# Autodesk Inventor assembly: buoy_mainboard
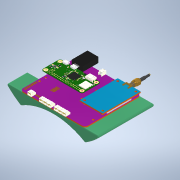
[picture p0: Inventor's stored thumbnail of the model, 180x180]
Saved by Autodesk Inventor 2020.2 (Build 242310000, 310)
## iProperties
Created: 2020-04-10
Part Number: buoy_mainboard
Document SubType Name: Assembly
Designer: agmlego
Mass: 108.257 g
Surface Area: 767.177 cm^2
Volume: 137.886 cm^3
Density: 0.785117 g/cm^3
Author: agmlego
## Documents named in this file (10)
- D:\projects\CreekFleet_AutoBuoy\Mechanical CAD\controls\buoy_mainboard.iam
- D:\projects\CreekFleet_AutoBuoy\Mechanical CAD\controls\buoy_pcb.ipt
- D:\projects\CreekFleet_AutoBuoy\Mechanical CAD\controls\pi-zero\RapberryPiZero.iam
- D:\projects\CreekFleet_AutoBuoy\Mechanical CAD\controls\XT09-SI.ipt
- D:\projects\CreekFleet_AutoBuoy\Mechanical CAD\controls\JST-PH-2\S2B-PH-K-S(LF)(SN)--3DModel-STEP-1.ipt
- D:\projects\CreekFleet_AutoBuoy\Mechanical CAD\controls\ND-105C.ipt
- D:\projects\CreekFleet_AutoBuoy\Mechanical CAD\controls\pololu\dual-g2-hpmd-18v18-24v14-raspberry-pi.ipt
- D:\projects\CreekFleet_AutoBuoy\Mechanical CAD\controls\mainboard_mount.ipt
- D:\projects\CreekFleet_AutoBuoy\Mechanical CAD\94459A140_BRASS HEAT-SET INSERT FOR PLASTIC.ipt
- D:\projects\CreekFleet_AutoBuoy\Mechanical CAD\controls\rp-sma_end.ipt
## Components (21 placed, 16 different names)
1. buoy_pcb:1 — Mate:1, Flush:1, Flush:2, Mate:2, Mate:3, Mate:4, Mate:5, Mate:6, Mate:7, Mate:8, Mate:9, Mate:10, Mate:11, Mate:12, Mate:13, Mate:14, Mate:15, Tangent:1, Tangent:2, Tangent:3, Tangent:4, Tangent:5, Tangent:6, Tangent:7, Tangent:8, Tangent:9, Tangent:10, Tangent:11, Tangent:12, Mate:19, Mate:20, Mate:21, Insert:1, Angle:1
2. RapberryPiZero:1 [sub-assembly] — Mate:2, Mate:3, Mate:4, Mate:16, Mate:17, Mate:18
3. XT09-SI:1 — Mate:5, Mate:6, Mate:7, Insert:8
4. CAN — Mate:15, Tangent:1, Tangent:2, Tangent:3
5. CURR — Mate:8, Flush:8, Tangent:4, Tangent:12
6. FLT — Mate:9, Flush:7, Flush:8, Tangent:11
7. SLP — Mate:10, Flush:6, Flush:7, Tangent:10
8. DIR — Mate:11, Flush:5, Flush:6, Tangent:9
9. PORT LED — Mate:12, Flush:4, Flush:5, Tangent:8
10. STAR LED — Mate:13, Flush:3, Flush:4, Tangent:7
11. ALLROUND LED — Mate:14, Flush:3, Tangent:5, Tangent:6
12. ND-105C:1 — Mate:16, Mate:17, Mate:18
13. dual-g2-hpmd-18v18-24v14-raspberry-pi:1 — Mate:19, Mate:20, Mate:21
14. mainboard_mount:1 — Insert:1, Angle:1, Insert:2, Insert:3, Insert:4, Insert:5, Insert:6, Insert:7
15. 94459A140_BRASS HEAT-SET INSERT FOR PLASTIC:1 — Insert:2
16. 94459A140_BRASS HEAT-SET INSERT FOR PLASTIC:2 — Insert:3
17. 94459A140_BRASS HEAT-SET INSERT FOR PLASTIC:3 — Insert:4
18. 94459A140_BRASS HEAT-SET INSERT FOR PLASTIC:4 — Insert:5
19. 94459A140_BRASS HEAT-SET INSERT FOR PLASTIC:5 — Insert:7
20. 94459A140_BRASS HEAT-SET INSERT FOR PLASTIC:6 — Insert:6
21. rp-sma_end:1 — Insert:8
## Relationships (50: Mate 21, Tangent 12, Flush 8, Insert 8, Angle 1)
- Mate:1: buoy_pcb:1
- Flush:1: buoy_pcb:1
- Flush:2: buoy_pcb:1
- Mate:2: buoy_pcb:1 ↔ RapberryPiZero:1
- Mate:3: buoy_pcb:1 ↔ RapberryPiZero:1
- Mate:4 (10 mm): buoy_pcb:1 ↔ RapberryPiZero:1
- Mate:5: buoy_pcb:1 ↔ XT09-SI:1
- Mate:6: buoy_pcb:1 ↔ XT09-SI:1
- Mate:7: buoy_pcb:1 ↔ XT09-SI:1
- Mate:8: buoy_pcb:1 ↔ CURR
- Mate:9: buoy_pcb:1 ↔ FLT
- Mate:10: buoy_pcb:1 ↔ SLP
- Mate:11: buoy_pcb:1 ↔ DIR
- Mate:12: buoy_pcb:1 ↔ PORT LED
- Mate:13: buoy_pcb:1 ↔ STAR LED
- Mate:14: buoy_pcb:1 ↔ ALLROUND LED
- Mate:15: buoy_pcb:1 ↔ CAN
- Tangent:1: buoy_pcb:1 ↔ CAN
- Tangent:2: buoy_pcb:1 ↔ CAN
- Tangent:3 (0.6 mm): buoy_pcb:1 ↔ CAN
- Flush:3: STAR LED ↔ ALLROUND LED
- Flush:4: PORT LED ↔ STAR LED
- Flush:5: DIR ↔ PORT LED
- Flush:6: SLP ↔ DIR
- Flush:7: FLT ↔ SLP
- Flush:8: CURR ↔ FLT
- Tangent:4: buoy_pcb:1 ↔ CURR
- Tangent:5: buoy_pcb:1 ↔ ALLROUND LED
- Tangent:6 (0.6 mm): buoy_pcb:1 ↔ ALLROUND LED
- Tangent:7 (0.6 mm): buoy_pcb:1 ↔ STAR LED
- Tangent:8 (0.6 mm): buoy_pcb:1 ↔ PORT LED
- Tangent:9 (0.6 mm): buoy_pcb:1 ↔ DIR
- Tangent:10 (0.6 mm): buoy_pcb:1 ↔ SLP
- Tangent:11 (0.6 mm): buoy_pcb:1 ↔ FLT
- Tangent:12 (0.6 mm): buoy_pcb:1 ↔ CURR
- Mate:16: RapberryPiZero:1 ↔ ND-105C:1
- Mate:17: RapberryPiZero:1 ↔ ND-105C:1
- Mate:18: RapberryPiZero:1 ↔ ND-105C:1
- Mate:19 (12 mm): buoy_pcb:1 ↔ dual-g2-hpmd-18v18-24v14-raspberry-pi:1
- Mate:20: buoy_pcb:1 ↔ dual-g2-hpmd-18v18-24v14-raspberry-pi:1
- Mate:21: buoy_pcb:1 ↔ dual-g2-hpmd-18v18-24v14-raspberry-pi:1
- Insert:1: buoy_pcb:1 ↔ mainboard_mount:1
- Angle:1 (0 deg): buoy_pcb:1 ↔ mainboard_mount:1
- Insert:2: mainboard_mount:1 ↔ 94459A140_BRASS HEAT-SET INSERT FOR PLASTIC:1
- Insert:3: mainboard_mount:1 ↔ 94459A140_BRASS HEAT-SET INSERT FOR PLASTIC:2
- Insert:4: mainboard_mount:1 ↔ 94459A140_BRASS HEAT-SET INSERT FOR PLASTIC:3
- Insert:5: mainboard_mount:1 ↔ 94459A140_BRASS HEAT-SET INSERT FOR PLASTIC:4
- Insert:6: mainboard_mount:1 ↔ 94459A140_BRASS HEAT-SET INSERT FOR PLASTIC:6
- Insert:7: mainboard_mount:1 ↔ 94459A140_BRASS HEAT-SET INSERT FOR PLASTIC:5
- Insert:8: XT09-SI:1 ↔ rp-sma_end:1
